# Autodesk Inventor assembly: CL3-100
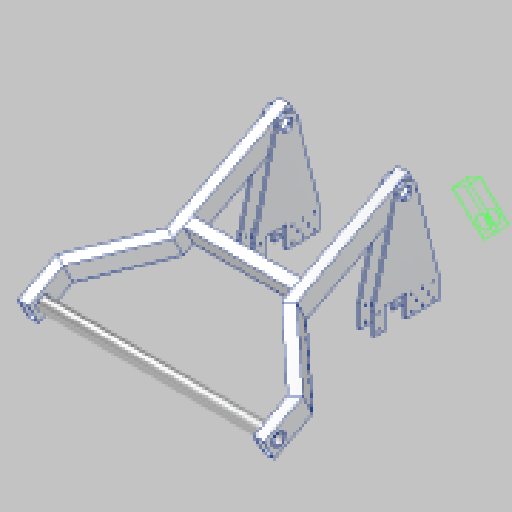
[picture p0: Inventor's stored thumbnail of the model, 512x512]
Saved by Autodesk Inventor 2023.5 (Build 275446000, 446)
## iProperties
Created: 2025-01-28
Part Number: CL3-100
Document SubType Name: Assembly
Designer: slick
Author: slick
## Documents named in this file (7)
- C:\Users\slick\OneDrive\Desktop\2025-ReefScape---CAD\Climber\CL3\CL3-100.iam
- C:\Users\slick\OneDrive\Desktop\2025-ReefScape---CAD\Climber\CL3\CL3-001.ipt
- C:\Users\slick\OneDrive\Desktop\2025-ReefScape---CAD\Climber\CL3\CL3-002.ipt
- C:\Users\slick\OneDrive\Desktop\2025-ReefScape---CAD\Climber\CL3\CL3-003.ipt
- C:\Users\slick\OneDrive\Desktop\2025-ReefScape---CAD\Climber\CL3\CL3-004.ipt
- C:\Users\slick\OneDrive\Desktop\2025-ReefScape---CAD\Climber\CL3\CL3-005.ipt
- C:\Users\slick\OneDrive\Desktop\2025-ReefScape---CAD\Climber\CL3\CL3-006.ipt
## Components (12 placed, 6 different names)
1. CL3-001:1 — Mate:1, Flush:1, Mate:2, Mate:9, Flush:5, Mate:10, Mate:11, Mate:15, Mate:16, Flush:10
2. CL3-002:1 — Mate:1, Flush:1, Mate:2, Flush:2, Mate:3, Mate:4
3. CL3-003:1 — Flush:2, Mate:3, Mate:4, Flush:6, Mate:19, Flush:11, Flush:12
4. CL3-001:2 — Mate:9, Flush:5, Mate:13, Mate:14, Mate:17, Mate:18
5. CL3-002:2
6. CL3-003:2 — Flush:6
7. CL3-004:1 — Flush:7, Mate:12, Mate:13, Flush:9, Mate:17
8. CL3-004:2 — Flush:7, Mate:10, Mate:15, Flush:8
9. CL3-004:3 — Mate:11, Mate:16, Flush:8
10. CL3-004:4 — Mate:12, Mate:14, Flush:9
11. CL3-005:1 — Flush:10, Mate:18, Flush:12
12. CL3-006:1 — Mate:19, Flush:11
## Relationships (31: Mate 19, Flush 12)
- Mate:1: CL3-001:1 ↔ CL3-002:1
- Flush:1: CL3-001:1 ↔ CL3-002:1
- Mate:2: CL3-001:1 ↔ CL3-002:1
- Flush:2: CL3-002:1 ↔ CL3-003:1
- Mate:3: CL3-002:1 ↔ CL3-003:1
- Mate:4: CL3-002:1 ↔ CL3-003:1
- [Mate]: CL3-001:2 ↔ CL3-002:2
- [Flush]: CL3-001:2 ↔ CL3-002:2
- [Mate]: CL3-001:2 ↔ CL3-002:2
- [Flush]: CL3-002:2 ↔ CL3-003:2
- [Mate]: CL3-002:2 ↔ CL3-003:2
- [Mate]: CL3-002:2 ↔ CL3-003:2
- Mate:9 (254 mm): CL3-001:1 ↔ CL3-001:2
- Flush:5: CL3-001:1 ↔ CL3-001:2
- Flush:6: CL3-003:1 ↔ CL3-003:2
- Flush:7: CL3-004:1 ↔ CL3-004:2
- Mate:10: CL3-001:1 ↔ CL3-004:2
- Mate:11: CL3-001:1 ↔ CL3-004:3
- Mate:12: CL3-004:1 ↔ CL3-004:4
- Mate:13: CL3-001:2 ↔ CL3-004:1
- Mate:14: CL3-001:2 ↔ CL3-004:4
- Mate:15: CL3-001:1 ↔ CL3-004:2
- Mate:16: CL3-001:1 ↔ CL3-004:3
- Flush:8: CL3-004:2 ↔ CL3-004:3
- Flush:9: CL3-004:1 ↔ CL3-004:4
- Mate:17: CL3-001:2 ↔ CL3-004:1
- Flush:10: CL3-001:1 ↔ CL3-005:1
- Mate:18: CL3-001:2 ↔ CL3-005:1
- Mate:19: CL3-003:1 ↔ CL3-006:1
- Flush:11: CL3-003:1 ↔ CL3-006:1
- Flush:12 (-254 mm): CL3-003:1 ↔ CL3-005:1
## Named parameters: d24_d18 = 0 mm, d25_d19 = 0 mm, d26_d20 = 0 mm, d27_d21 = 0 mm, d28_d22 = 0 mm, d29_d23 = 0 mm
